# Autodesk Inventor assembly: MPPC
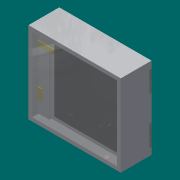
[picture p0: Inventor's stored thumbnail of the model, 180x180]
Saved by Autodesk Inventor 2016 SP1 (Build 200210100, 210)
## iProperties
Created: 2016-02-09
Part Number: MPPC
Document SubType Name: Assembly
Designer: Sawaiz
Author: Sawaiz
## Documents named in this file (3)
- C:\Users\sawaiz\OneDrive\projects\inventorLibrary\MPPC\3x3\13360-30xxPE\13360-30xxPE.iam
- C:\Users\sawaiz\OneDrive\projects\inventorLibrary\MPPC\3x3\13360-30xxPE\mppc.ipt
- C:\Users\sawaiz\OneDrive\projects\inventorLibrary\MPPC\3x3\13360-30xxPE\lens.ipt
## Components (2 placed, 2 different names)
1. mppc:1 — Flush:1
2. lens:1 — Flush:1
## Relationships (1: Flush 1)
- Flush:1: mppc:1 ↔ lens:1
